# Autodesk Inventor assembly: Pick_&_Place_Complete_Assembly
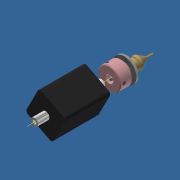
[picture p0: Inventor's stored thumbnail of the model, 180x180]
Saved by Autodesk Inventor 2015 (Build 190159000, 159)
## iProperties
Created: 2015-01-06
Part Number: Pick_&_Place_Complete_Assembly
Document SubType Name: Assembly
Designer: ice
Author: ice
## Documents named in this file (4)
- C:\Users\ice\Documents\GitHub\PnP-Magnetic-Tool-Tip\Inventor\Pick_&_Place_Complete_Assembly_Minimalist_Extender.iam
- C:\Users\ice\Documents\GitHub\PnP-Magnetic-Tool-Tip\Inventor\Extender_Minimalist_Assembly.iam
- C:\Users\ice\Documents\GitHub\PnP-Magnetic-Tool-Tip\Inventor\Nozzle_Assembly_Rev_A.iam
- C:\Users\ice\Documents\GitHub\PnP-Magnetic-Tool-Tip\Inventor\NEMA8.ipt
## Components (3 placed, 3 different names)
1. Extender_Minimalist_Assembly:1 [sub-assembly] — Mate:1, Mate:2, Mate:3
2. Nozzle_Assembly_Rev_A:1 [sub-assembly] — Mate:1, Mate:2
3. NEMA8:1 — Mate:3
## Relationships (3: Mate 3)
- Mate:1: Extender_Minimalist_Assembly:1 ↔ Nozzle_Assembly_Rev_A:1
- Mate:2: Extender_Minimalist_Assembly:1 ↔ Nozzle_Assembly_Rev_A:1
- Mate:3: Extender_Minimalist_Assembly:1 ↔ NEMA8:1
